# Autodesk Inventor assembly: gear_MIR
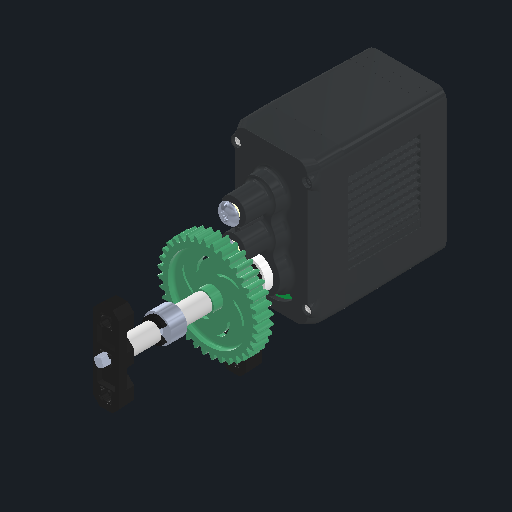
[picture p0: Inventor's stored thumbnail of the model, 512x512]
Saved by Autodesk Inventor 2024 (Build 280153000, 153)
## iProperties
Created: 2023-08-09
Part Number: gear_MIR
Document SubType Name: Assembly
Designer: macbook
Author: macbook
## Documents named in this file (14)
- \\Mac\Home\Desktop\code\1599V-VRC\Cad\Assembly\v4\gear_MIR.iam
- \\Mac\Home\Desktop\code\1599V-VRC\Cad\Motion\Gears\LS 36T Gear_MIR8.ipt
- \\Mac\Home\Desktop\code\1599V-VRC\Cad\Motion\Shaft LS\Shaft LS\Shaft LS 3.0.ipt
- \\Mac\Home\Desktop\code\1599V-VRC\Cad\Motion\Shaft LS\Shaft LS.ipt
- \\Mac\Home\Desktop\code\1599V-VRC\Cad\Electronics\Motors with Screws\AluM-StarS_MIR8.iam
- \\Mac\Home\Desktop\code\1599V-VRC\Cad\Motion\Spacers\Washer Teflon\TWasher .375 OD x .03125.ipt
- \\Mac\Home\Desktop\code\1599V-VRC\Cad\Motion\Spacers\Washer Teflon.ipt
- \\Mac\Home\Desktop\code\1599V-VRC\Cad\Motion\Shaft LS\Bearing Flat_MIR8.ipt
- \\Mac\Home\Desktop\code\1599V-VRC\Cad\Motion\Spacers\Spacer Nylon .500 OD\NSpacer White .500 OD x .125.ipt
- \\Mac\Home\Desktop\code\1599V-VRC\Cad\Motion\Spacers\Spacer Nylon .500 OD.ipt
- \\Mac\Home\Desktop\code\1599V-VRC\Cad\Assembly\12mm spacer_MIR.ipt
- \\Mac\Home\Desktop\code\1599V-VRC\Cad\Motion\Shaft LS\Shaft Collar Metal\Shaft Collar Set Screw_MIR7.iam
- \\Mac\Home\Desktop\code\1599V-VRC\Cad\Motion\Spacers\Spacer Nylon Click On\Nspacer Click On x .0625.ipt
- \\Mac\Home\Desktop\code\1599V-VRC\Cad\Motion\Spacers\Spacer Nylon Click On.ipt
## Components (11 placed, 9 different names)
1. LS 36T Gear_MIR8:1 — Insert:1, Insert:23
2. Shaft LS 3.0:1 — Mate:1
3. AluM-StarS_MIR8:1 [sub-assembly] — Mate:1, Flush:1, Insert:20
4. TWasher .375 OD x .03125:1 — Insert:17, Insert:1
5. Bearing Flat_MIR8:1 — Flush:1, Insert:19, Insert:21, Insert:17
6. NSpacer White .500 OD x .125:1 — Insert:19
7. Bearing Flat_MIR8:2 — Insert:21, Insert:20, Insert:22
8. 12mm spacer_MIR:1 — Insert:22
9. Shaft Collar Set Screw_MIR7:1 [sub-assembly] — Insert:24, Insert:25
10. 12mm spacer_MIR:2 — Insert:24, Insert:23
11. Nspacer Click On x .0625:1 — Insert:25
## Relationships (11: Insert 9, Mate 1, Flush 1)
- Mate:1: Shaft LS 3.0:1 ↔ AluM-StarS_MIR8:1
- Flush:1: AluM-StarS_MIR8:1 ↔ Bearing Flat_MIR8:1
- Insert:19: Bearing Flat_MIR8:1 ↔ NSpacer White .500 OD x .125:1
- Insert:21 (44.45 mm): Bearing Flat_MIR8:1 ↔ Bearing Flat_MIR8:2
- Insert:20 (42.8625 mm): AluM-StarS_MIR8:1 ↔ Bearing Flat_MIR8:2
- Insert:17 (1.5875 mm): TWasher .375 OD x .03125:1 ↔ Bearing Flat_MIR8:1
- Insert:1: LS 36T Gear_MIR8:1 ↔ TWasher .375 OD x .03125:1
- Insert:22: Bearing Flat_MIR8:2 ↔ 12mm spacer_MIR:1
- Insert:24: Shaft Collar Set Screw_MIR7:1 ↔ 12mm spacer_MIR:2
- Insert:23: LS 36T Gear_MIR8:1 ↔ 12mm spacer_MIR:2
- Insert:25: Shaft Collar Set Screw_MIR7:1 ↔ Nspacer Click On x .0625:1
